# Autodesk Inventor assembly: wheeldblsprocket
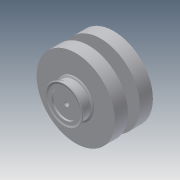
[picture p0: Inventor's stored thumbnail of the model, 180x180]
Saved by Autodesk Inventor 2014 (Build 180170000, 170)
## iProperties
Created: 2016-01-12
Part Number: wheeldblsprocket
Document SubType Name: Assembly
Designer: Paul
Author: Paul
## Documents named in this file (3)
- C:\Users\Paul\Documents\Inventor\first 2016\wheeldblsprocket.iam
- C:\Users\Paul\Documents\Inventor\first 2016\wheel.ipt
- C:\Users\Paul\Documents\Inventor\first 2016\sprocket.ipt
## Components (6 placed, 2 different names)
1. wheel:1 — Mate:5, Mate:6
2. wheel:2 — Mate:7, Mate:8, Mate:9, Mate:10
3. sprocket:1 — Mate:1, Mate:3, Mate:10
4. sprocket:2 — Mate:2, Mate:4, Mate:6, Mate:7, Mate:8
5. sprocket:3 — Mate:2, Mate:4, Mate:5
6. sprocket:4 — Mate:1, Mate:3, Mate:9
## Relationships (10: Mate 10)
- Mate:1: sprocket:1 ↔ sprocket:4
- Mate:2: sprocket:2 ↔ sprocket:3
- Mate:3: sprocket:1 ↔ sprocket:4
- Mate:4: sprocket:2 ↔ sprocket:3
- Mate:5: wheel:1 ↔ sprocket:3
- Mate:6: wheel:1 ↔ sprocket:2
- Mate:7: wheel:2 ↔ sprocket:2
- Mate:8: wheel:2 ↔ sprocket:2
- Mate:9: wheel:2 ↔ sprocket:4
- Mate:10: wheel:2 ↔ sprocket:1
